# Autodesk Inventor assembly: hoops_sml_med_lrg
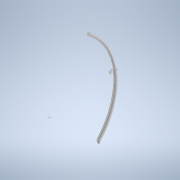
[picture p0: Inventor's stored thumbnail of the model, 180x180]
Saved by Autodesk Inventor 2021 (Build 250183000, 183)
## iProperties
Created: 2021-05-05
Part Number: hoops_sml_med_lrg
Document SubType Name: Assembly
## Documents named in this file (9)
- C:\Users\ocon0143\OneDrive - Flinders\Advn Mech Design Shared\6_Development\2_Design\inventor\hoop_slider\hoops_sml_med_lrg.iam
- C:\Users\ocon0143\OneDrive - Flinders\Advn Mech Design Shared\6_Development\2_Design\inventor\hoop_slider\large_hoop.ipt
- C:\Users\ocon0143\OneDrive - Flinders\Advn Mech Design Shared\6_Development\2_Design\inventor\hoop_slider\medium_hoop.ipt
- C:\Users\ocon0143\OneDrive - Flinders\Advn Mech Design Shared\6_Development\2_Design\inventor\rack_pinion\pinion.ipt
- C:\Users\ocon0143\OneDrive - Flinders\Advn Mech Design Shared\6_Development\2_Design\inventor\hoop_slider\small_hoop.ipt
- C:\Users\ocon0143\OneDrive - Flinders\Advn Mech Design Shared\6_Development\2_Design\inventor\rack_pinion\tooth.ipt
- C:\Users\ocon0143\OneDrive - Flinders\Advn Mech Design Shared\6_Development\2_Design\inventor\rack_pinion\pulley_guide.ipt
- C:\Users\ocon0143\OneDrive - Flinders\Advn Mech Design Shared\6_Development\2_Design\inventor\rack_pinion\large_bearings.ipt
- C:\Users\ocon0143\OneDrive - Flinders\Advn Mech Design Shared\6_Development\2_Design\inventor\rack_pinion\medium_bearings.ipt
## Components (67 placed, 8 different names)
1. large_hoop:1 — Mate:1, Flush:1, Flush:12
2. medium_hoop:1 — Mate:2, Flush:2, Mate:4, Flush:8, Flush:9, Mate:6, Mate:7
3. pinion:1 — Flush:6
4. small_hoop:1 — Mate:3, Flush:7, Flush:10, Mate:5, Flush:11
5. pulley_guide:1 — Flush:10, Mate:5, Flush:11
6. large_bearings:1 — Mate:6, Flush:12
7. medium_bearings:1 — Flush:13, Mate:7
8. tooth:1 — Mate:4, Flush:8, Flush:9
9. tooth:2
10. tooth:3
11. tooth:4
12. tooth:5
13. tooth:6
14. tooth:7
15. tooth:8
16. tooth:9
17. tooth:10
18. tooth:11
19. tooth:12
20. tooth:13
21. tooth:14
22. tooth:15
23. tooth:16
24. tooth:17
25. tooth:18
26. tooth:19
27. tooth:20
28. tooth:21
29. tooth:22
30. tooth:23
31. tooth:24
32. tooth:25
33. tooth:26
34. tooth:27
35. tooth:28
36. tooth:29
37. tooth:30
38. tooth:31
39. tooth:32
40. tooth:33
41. tooth:34
42. tooth:35
43. tooth:36
44. tooth:37
45. tooth:38
46. tooth:39
47. tooth:40
48. tooth:41
49. tooth:42
50. tooth:43
51. tooth:44
52. tooth:45
53. tooth:46
54. tooth:47
55. tooth:48
56. tooth:49
57. tooth:50
58. tooth:51
59. tooth:52
60. tooth:53
61. tooth:54
62. tooth:55
63. tooth:56
64. tooth:57
65. tooth:58
66. tooth:59
67. tooth:60
## Component patterns: (60 elements, first: tooth:1)
## Relationships (17: Flush 10, Mate 7)
- Mate:1: large_hoop:1
- Mate:2: medium_hoop:1
- Flush:1: large_hoop:1
- Flush:2: medium_hoop:1
- Flush:6: pinion:1
- Mate:3: small_hoop:1
- Flush:7: small_hoop:1
- Mate:4: medium_hoop:1 ↔ tooth:1
- Flush:8: medium_hoop:1 ↔ tooth:1
- Flush:9: medium_hoop:1 ↔ tooth:1
- Flush:10 (4 mm): small_hoop:1 ↔ pulley_guide:1
- Mate:5 (1622 mm): small_hoop:1 ↔ pulley_guide:1
- Flush:11: small_hoop:1 ↔ pulley_guide:1
- Mate:6: medium_hoop:1 ↔ large_bearings:1
- Flush:12: large_hoop:1 ↔ large_bearings:1
- Flush:13: medium_bearings:1
- Mate:7: medium_hoop:1 ↔ medium_bearings:1
